# Autodesk Inventor assembly: Tool_Head
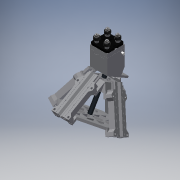
[picture p0: Inventor's stored thumbnail of the model, 180x180]
Saved by Autodesk Inventor 2019 (Build 230136000, 136)
## iProperties
Created: 2021-01-18
Part Number: Tool_Head
Document SubType Name: Assembly
Designer: zhanb
Author: zhanb
## Documents named in this file (9)
- F:\3D Objects\Inventor\Coursework\ECE HyperRail\Tool_Head_Assem.iam
- F:\3D Objects\Inventor\Coursework\ECE HyperRail\Pen_Holder_Assem.iam
- F:\3D Objects\Inventor\Coursework\ECE HyperRail\4-Tool_Lower.ipt
- F:\3D Objects\Inventor\Coursework\ECE HyperRail\4-Tool_Upper.ipt
- F:\3D Objects\Inventor\Coursework\ECE HyperRail\Stock Parts\.375_HexShaft.ipt
- F:\3D Objects\Inventor\Coursework\ECE HyperRail\Gantry\Mini V Gantry Kit.iam
- F:\3D Objects\Inventor\Coursework\ECE HyperRail\Gantry_Mount_Rail.ipt
- F:\3D Objects\Inventor\Coursework\ECE HyperRail\Gantry_Mount.ipt
- F:\3D Objects\Inventor\Coursework\ECE HyperRail\Stock Parts\Release_Pin.ipt
## Components (11 placed, 8 different names)
1. Mini V Gantry Kit:1 [sub-assembly] — Mate:11, Mate:12, Flush:14, Mate:13, Mate:14, Mate:15
2. Gantry_Mount_Rail:1 — Mate:13, Mate:14, Mate:15, Mate:16, Mate:17
3. Gantry_Mount:1 — Mate:16, Mate:17, Mate:18, Mate:19, Mate:20, Angle:1
4. 4-Tool_Upper:1 — Mate:2, Flush:8, Flush:9, Flush:10, Flush:11, Flush:12, Mate:3, Mate:9, Mate:10, Mate:19, Mate:20
5. 4-Tool_Lower:1 — Flush:8, Flush:9, Flush:10, Flush:11, Flush:12, Mate:4, Flush:13
6. Release_Pin:1 — Mate:18
7. .375_HexShaft:1 — Mate:9, Mate:10, Flush:13
8. Pen_Holder_Assem:1 [sub-assembly] — Mate:2, Mate:3, Mate:4
9. Pen_Holder_Assem:2 [sub-assembly] — Angle:1
10. Pen_Holder_Assem:3 [sub-assembly]
11. Pen_Holder_Assem:4 [sub-assembly]
## Component patterns: (4 elements, first: Pen_Holder_Assem:1)
## Relationships (23: Mate 15, Flush 7, Angle 1)
- Mate:2: 4-Tool_Upper:1 ↔ Pen_Holder_Assem:1
- Flush:8: 4-Tool_Upper:1 ↔ 4-Tool_Lower:1
- Flush:9: 4-Tool_Upper:1 ↔ 4-Tool_Lower:1
- Flush:10: 4-Tool_Upper:1 ↔ 4-Tool_Lower:1
- Flush:11: 4-Tool_Upper:1 ↔ 4-Tool_Lower:1
- Flush:12: 4-Tool_Upper:1 ↔ 4-Tool_Lower:1
- Mate:3: 4-Tool_Upper:1 ↔ Pen_Holder_Assem:1
- Mate:4: 4-Tool_Lower:1 ↔ Pen_Holder_Assem:1
- Mate:9: 4-Tool_Upper:1 ↔ .375_HexShaft:1
- Mate:10: 4-Tool_Upper:1 ↔ .375_HexShaft:1
- Flush:13 (-6.35 mm): 4-Tool_Lower:1 ↔ .375_HexShaft:1
- Mate:11: Mini V Gantry Kit:1
- Mate:12: Mini V Gantry Kit:1
- Flush:14: Mini V Gantry Kit:1
- Mate:13: Mini V Gantry Kit:1 ↔ Gantry_Mount_Rail:1
- Mate:14: Mini V Gantry Kit:1 ↔ Gantry_Mount_Rail:1
- Mate:15: Mini V Gantry Kit:1 ↔ Gantry_Mount_Rail:1
- Mate:16 (0.1984 mm): Gantry_Mount_Rail:1 ↔ Gantry_Mount:1
- Mate:17: Gantry_Mount_Rail:1 ↔ Gantry_Mount:1
- Mate:18: Gantry_Mount:1 ↔ Release_Pin:1
- Mate:19: Gantry_Mount:1 ↔ 4-Tool_Upper:1
- Mate:20 (12.7 mm): Gantry_Mount:1 ↔ 4-Tool_Upper:1
- Angle:1 (0 deg): Gantry_Mount:1 ↔ Pen_Holder_Assem:2
